# Autodesk Inventor assembly: Galileo Clockwork
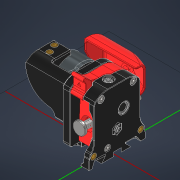
[picture p0: Inventor's stored thumbnail of the model, 180x180]
Saved by Autodesk Inventor 2022.2 (Build 262287010, 287A)
## iProperties
Created: 2022-03-15
Part Number: Galileo Clockwork
Document SubType Name: Assembly
Designer: sleib
Author: sleib
## Documents named in this file (14)
- C:\Users\sleib\Projekte\Voron-2\CAD\Inventor\Galileo Clockwork\Galileo Clockwork.iam
- C:\Users\sleib\Projekte\Voron-2\CAD\Inventor\Galileo Clockwork\Galileo Chain Anchor China.iam
- C:\Users\sleib\Projekte\Voron-2\CAD\Inventor\Galileo Clockwork\Galileo Extruder.iam
- C:\Users\sleib\Projekte\Voron-2\CAD\Inventor\Galileo Clockwork\Galileo Plate.iam
- C:\Users\sleib\Projekte\Voron-2\CAD\Inventor\Galileo Clockwork\Galileo Body.iam
- C:\Users\sleib\Projekte\Voron-2\CAD\Inventor\Galileo Clockwork\Galileo Guide.iam
- C:\Users\sleib\Projekte\Voron-2\CAD\Inventor\Galileo Clockwork\Shuttle.ipt
- C:\Users\sleib\Projekte\Voron-2\CAD\Inventor\M3x25 SHCS.ipt
- C:\Users\sleib\Projekte\Voron-2\CAD\Inventor\M3x30 SHCS.ipt
- C:\Users\sleib\Projekte\Voron-2\CAD\Inventor\M3x8 SHCS.ipt
- C:\Users\sleib\Projekte\Voron-2\CAD\Inventor\M3x14 SHCS.ipt
- C:\Users\sleib\Projekte\Voron-2\CAD\Inventor\M3x10 SHCS.ipt
- C:\Users\sleib\Projekte\Voron-2\CAD\Inventor\Galileo Clockwork\Top Latch Coupler.ipt
- C:\Users\sleib\Projekte\Voron-2\CAD\Inventor\Galileo Clockwork\Wire Cover.ipt
## Components (15 placed, 13 different names)
1. Galileo Body:1 [sub-assembly] — Passend:6, Passend:7, Passend:8, Passend:9, Passend:10, Passend:11, Passend:12, Passend:18, Passend:19, Winkel:1, Passend:20, Passend:21, Passend:22, Passend:23, Passend:24, Passend:25, Passend:35, Passend:36, Passend:37, Passend:38, Passend:39
2. Galileo Plate:1 [sub-assembly] — Passend:10, Passend:11, Passend:12, Passend:15, Passend:16, Passend:17, Passend:28, Passend:29, Passend:32, Passend:33, Passend:42, Passend:43, Passend:44
3. Galileo Extruder:1 [sub-assembly] — Passend:42, Passend:43, Passend:44
4. Galileo Guide:1 [sub-assembly] — Passend:6, Passend:7, Tangential:2
5. Galileo Chain Anchor China:1 [sub-assembly] — Passend:15, Passend:16, Passend:17, Passend:30, Passend:31
6. Top Latch Coupler:1 — Passend:35, Tangential:3, Passend:36
7. Shuttle:1 — Passend:8, Passend:9, Tangential:2, Tangential:3
8. Wire Cover:1 — Passend:37, Passend:38, Passend:40, Passend:41
9. M3x25 SHCS:1 — Passend:20, Passend:21
10. M3x30 SHCS:1 — Passend:24, Passend:25
11. M3x25 SHCS:2 — Passend:22, Passend:23
12. M3x8 SHCS:1 — Passend:39, Passend:40
13. M3x14 SHCS:1 — Passend:28, Passend:29, Passend:41
14. M3x10 SHCS:1 — Passend:30, Passend:31
15. M3x14 SHCS:2 — Passend:32, Passend:33
## Relationships (37: Mate 34, Tangent 2, Angle 1)
- Passend:6 [Mate]: Galileo Body:1 ↔ Galileo Guide:1
- Passend:7 [Mate]: Galileo Body:1 ↔ Galileo Guide:1
- Passend:8 [Mate]: Galileo Body:1 ↔ Shuttle:1
- Passend:9 [Mate]: Galileo Body:1 ↔ Shuttle:1
- Passend:10 [Mate]: Galileo Body:1 ↔ Galileo Plate:1
- Passend:11 [Mate]: Galileo Body:1 ↔ Galileo Plate:1
- Passend:12 [Mate]: Galileo Body:1 ↔ Galileo Plate:1
- Passend:15 [Mate]: Galileo Plate:1 ↔ Galileo Chain Anchor China:1
- Passend:16 [Mate]: Galileo Plate:1 ↔ Galileo Chain Anchor China:1
- Passend:17 [Mate]: Galileo Plate:1 ↔ Galileo Chain Anchor China:1
- Passend:18 [Mate]: Galileo Body:1
- Passend:19 [Mate]: Galileo Body:1
- Winkel:1 [Angle] (0 deg): Galileo Body:1
- Tangential:2: Galileo Guide:1 ↔ Shuttle:1
- Passend:20 [Mate]: Galileo Body:1 ↔ M3x25 SHCS:1
- Passend:21 [Mate]: Galileo Body:1 ↔ M3x25 SHCS:1
- Passend:22 [Mate]: Galileo Body:1 ↔ M3x25 SHCS:2
- Passend:23 [Mate]: Galileo Body:1 ↔ M3x25 SHCS:2
- Passend:24 [Mate]: Galileo Body:1 ↔ M3x30 SHCS:1
- Passend:25 [Mate]: Galileo Body:1 ↔ M3x30 SHCS:1
- Passend:28 [Mate]: Galileo Plate:1 ↔ M3x14 SHCS:1
- Passend:29 [Mate]: Galileo Plate:1 ↔ M3x14 SHCS:1
- Passend:30 [Mate]: Galileo Chain Anchor China:1 ↔ M3x10 SHCS:1
- Passend:31 [Mate]: Galileo Chain Anchor China:1 ↔ M3x10 SHCS:1
- Passend:32 [Mate]: Galileo Plate:1 ↔ M3x14 SHCS:2
- Passend:33 [Mate]: Galileo Plate:1 ↔ M3x14 SHCS:2
- Passend:35 [Mate]: Galileo Body:1 ↔ Top Latch Coupler:1
- Tangential:3: Top Latch Coupler:1 ↔ Shuttle:1
- Passend:36 [Mate]: Galileo Body:1 ↔ Top Latch Coupler:1
- Passend:37 [Mate]: Galileo Body:1 ↔ Wire Cover:1
- Passend:38 [Mate]: Galileo Body:1 ↔ Wire Cover:1
- Passend:39 [Mate]: Galileo Body:1 ↔ M3x8 SHCS:1
- Passend:40 [Mate]: Wire Cover:1 ↔ M3x8 SHCS:1
- Passend:41 [Mate]: Wire Cover:1 ↔ M3x14 SHCS:1
- Passend:42 [Mate]: Galileo Plate:1 ↔ Galileo Extruder:1
- Passend:43 [Mate]: Galileo Plate:1 ↔ Galileo Extruder:1
- Passend:44 [Mate]: Galileo Plate:1 ↔ Galileo Extruder:1
